# Autodesk Inventor assembly: Lever
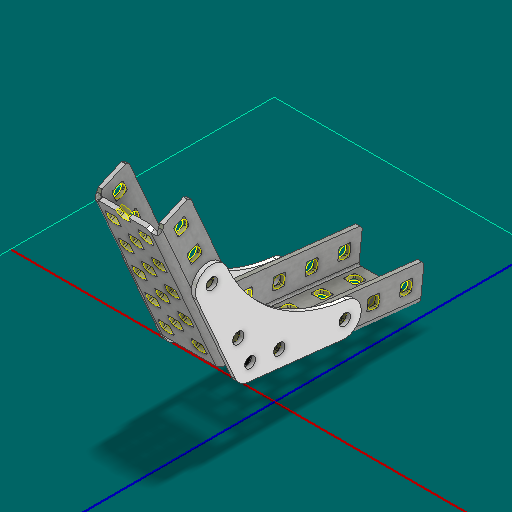
[picture p0: Inventor's stored thumbnail of the model, 512x512]
Saved by Autodesk Inventor 2025 (Build 290162000, 162)
## iProperties
Created: 2024-10-22
Part Number: Lever
Document SubType Name: Assembly
Designer: averey
Author: averey
## Documents named in this file (5)
- C:\Users\avere\VEX\High Stakes\CAD\V2\Clamp\Lever.iam
- C:\Users\avere\VEX\High Stakes\CAD\ROBOPROS-CAD-Inventor\Structure\C Channel\Aluminum 1x2x1\Alu C 1x2x1x5.ipt
- C:\Users\avere\VEX\High Stakes\CAD\V2\Clamp\Custom Parts\60 Degree Gusset.ipt
- C:\Users\avere\VEX\High Stakes\CAD\ROBOPROS-CAD-Inventor\Structure\Standoff\Standoff 1.00.ipt
- C:\Users\avere\VEX\High Stakes\CAD\ROBOPROS-CAD-Inventor\Structure\Standoff.ipt
## Components (5 placed, 3 different names)
1. Alu C 1x2x1x5:1 — Insert:1, Mate:2, Mate:4
2. Alu C 1x2x1x5:2 — Insert:2, Mate:1, Insert:3, Mate:3
3. 60 Degree Gusset:1 — Insert:1, Insert:2, Mate:1, Mate:2, Mate:5
4. 60 Degree Gusset:2 — Insert:3, Mate:3, Mate:4, Insert:4
5. Standoff 1.00:1 — Insert:4, Mate:5
## Relationships (9: Mate 5, Insert 4)
- Insert:1: Alu C 1x2x1x5:1 ↔ 60 Degree Gusset:1
- Insert:2: Alu C 1x2x1x5:2 ↔ 60 Degree Gusset:1
- Mate:1: Alu C 1x2x1x5:2 ↔ 60 Degree Gusset:1
- Mate:2: Alu C 1x2x1x5:1 ↔ 60 Degree Gusset:1
- Insert:3: Alu C 1x2x1x5:2 ↔ 60 Degree Gusset:2
- Mate:3: Alu C 1x2x1x5:2 ↔ 60 Degree Gusset:2
- Mate:4: Alu C 1x2x1x5:1 ↔ 60 Degree Gusset:2
- Insert:4: 60 Degree Gusset:2 ↔ Standoff 1.00:1
- Mate:5: 60 Degree Gusset:1 ↔ Standoff 1.00:1
